# Autodesk Inventor assembly: RBID6
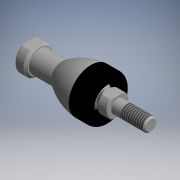
[picture p0: Inventor's stored thumbnail of the model, 180x180]
Saved by Autodesk Inventor 2017.3 (Build 213256000, 256)
## iProperties
Category: PARTsolutions
Company: MISUMI
Part Number: RBID6
Catalog Web Link: www.cadenas.de
Description: RBID, RBIDL-Rod End Bearings - Link Ball Type with Thread - Link Ball Straight Type
Vendor: MISUMI
Document SubType Name: Assembly
Designer: partserver
Manufacturer: MISUMI
Mass: 6.891 g
Surface Area: 38.6859 cm^2
Volume: 6.891 cm^3
Density: 1 g/cm^3
Title: RBID6
Author: Cadenas PARTsolutions
Comments: Rod End Bearings - Link Ball Type with Thread - Link Ball Straight Type
PSOL_IDENT_0: {$CADENAS_DATA\23d-libs\misumi\metric\34_cylinders\rbid_asmtab.prj},166 {VTYP=3D},{STYP=ASSTAB},{NB=
PSOL_IDENT_1: RBID6},{LINA=RBID6},{NN=RBID, RBIDL},{DATE=30.06.2021 13:14:17},{GEOMDATE=04.07.2011},{VERSION=},{LI
PSOL_IDENT_2: NEID=20},{WBVAR=TRS,MP},{WBNUMERIC=}  {NB=RBID6},{LINA=RBID6},{KT=DUMMY},{PN=RBID6},{TYPE=RBID},{TRS=
PSOL_IDENT_3: 1},{TRS1='1', 'Right-Hand Thread', '2', 'Left-Hand Thread'},{MATH=High Strength Zinc Alloy},{MATS=10
PSOL_IDENT_4: 35 Steel},{HARDS=20~28HRC},{MATB=NBR Type Special Synthetic Rubber},{HARD=Sphere 650HV~},{M=6},{D=10
PSOL_IDENT_5: .0},{D1=13},{D2=20},{L=55.2},{L1=28},{L2=15},{MP=1},{MPA='1','M6x1.0'},{L3=5.0},{W=11},{DD=6},{DDTOL=
PSOL_IDENT_6: 0/-0.030},{LL=27.2},{LL1=12.2},{LL2=11},{W1=8},{D3=10},{D4=20},{BD=12.700},{ASF=25},{PK=3730},{SLCT=
PSOL_IDENT_7: 7450},{SLCC=14900},{MASS=40},{NDM=6},{P=1},{KDM=4.917},{PPATH=rbid_templ.prj},{RCS=0.03 or Less},{AC
PSOL_IDENT_8: S=0.1 or Less}
NB: RBID6
NN: RBID, RBIDL
NT: Rod End Bearings - Link Ball Type with Thread - Link Ball Straight Type
NBSYN: $PN.
LINA: RBID6
CATALOG: Misumi
PN: RBID6
TRS: Right-Hand Thread
MATH: High Strength Zinc Alloy
MATS: 1035 Steel
HARDS: 20~28HRC
MATB: NBR Type Special Synthetic Rubber
HARD: Sphere 650HV~
M: 6
D: 10
D1: 13
D2: 20
L: 55.2
L1: 28
L2: 15
MP: M6x1.0
L3: 5
W: 11
DD: 6
DDTOL: 0/-0.030
LL: 27.2
LL1: 12.2
LL2: 11
W1: 8
D3: 10
D4: 20
BD: 12.7
ASF: 25
PK: 3730
SLCT: 7450
SLCC: 14900
MASS: 40
RCS: 0.03 or Less
ACS: 0.1 or Less
SUPPLIER: MISUMI
ARTICLENO: RBID6
BOMINFO: RBID6
CREATOR: CADENAS GmbH
## Documents named in this file (4)
- e:\temp\worker_28\temp\exporttempdir_4800_114_n0Mkt\format_0\RBID6.iam
- e:\temp\worker_28\temp\exporttempdir_4800_114_n0Mkt\format_0\RBID6dummy.ipt
- e:\temp\worker_28\temp\exporttempdir_4800_114_n0Mkt\format_0\RBID6holder.ipt
- e:\temp\worker_28\temp\exporttempdir_4800_114_n0Mkt\format_0\RBID6shank.ipt
## Components (3 placed, 3 different names)
1. RBID6dummy:1 — dummy_XY@1 <-> holder_XY@2, dummy_Z@1 <-> holder_Z@2, dummy_YZ@1 <-> holder_YZ@2
2. RBID6holder:1 — dummy_XY@1 <-> holder_XY@2, dummy_Z@1 <-> holder_Z@2, dummy_YZ@1 <-> holder_YZ@2, holder_XY@2 <-> shank_XY@3, holder_Z@2 <-> shank_Z@3
3. RBID6shank:1 — holder_XY@2 <-> shank_XY@3, holder_Z@2 <-> shank_Z@3
## Relationships (5: Mate 4, Angle 1)
- dummy_XY@1 <-> holder_XY@2 [Mate]: RBID6dummy:1 ↔ RBID6holder:1
- dummy_Z@1 <-> holder_Z@2 [Mate]: RBID6dummy:1 ↔ RBID6holder:1
- dummy_YZ@1 <-> holder_YZ@2 [Angle] (0 deg): RBID6dummy:1 ↔ RBID6holder:1
- holder_XY@2 <-> shank_XY@3 [Mate]: RBID6holder:1 ↔ RBID6shank:1
- holder_Z@2 <-> shank_Z@3 [Mate]: RBID6holder:1 ↔ RBID6shank:1
